# Autodesk Inventor assembly: KitBot-Obr
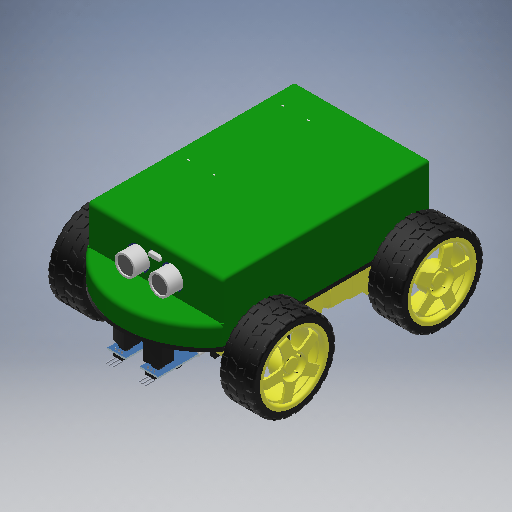
[picture p0: Inventor's stored thumbnail of the model, 512x512]
Saved by Autodesk Inventor 2025.1 (Build 291241020, 241B)
## iProperties
Created: 2024-12-26
Part Number: KitBot-Obr
Document SubType Name: Assembly
Designer: 53433618895
Author: 53433618895
## Documents named in this file (10)
- C:\Users\53433618895\OneDrive - SESISENAISP - Corporativo\FRC\2025\OBR\KitBot-Obr.iam
- C:\Users\53433618895\OneDrive - SESISENAISP - Corporativo\FRC\2025\OBR\tampa obr.ipt
- C:\Users\53433618895\OneDrive - SESISENAISP - Corporativo\FRC\2025\OBR\BASE.ipt
- C:\Users\53433618895\OneDrive - SESISENAISP - Corporativo\FRC\2025\OBR\arduino uno.iam
- C:\Users\53433618895\OneDrive - SESISENAISP - Corporativo\FRC\2025\OBR\Battery Holder ASSY V2.iam
- C:\Users\53433618895\OneDrive - SESISENAISP - Corporativo\FRC\2025\OBR\HCSR04 Ultrasonic Sensor.ipt
- C:\Users\53433618895\OneDrive - SESISENAISP - Corporativo\FRC\2025\OBR\infravermelho.ipt
- C:\Users\53433618895\OneDrive - SESISENAISP - Corporativo\FRC\2025\OBR\dc_motor_and_wheel.ipt
- C:\Users\53433618895\OneDrive - SESISENAISP - Corporativo\FRC\2025\OBR\Ponte H.ipt
- C:\Users\53433618895\OneDrive - SESISENAISP - Corporativo\FRC\2025\OBR\protobord.ipt
## Components (13 placed, 9 different names)
1. tampa obr:1 — Alinhado:1, Coincidente:10, Coincidente:26, Coincidente:27, Coincidente:28, Coincidente:40, Coincidente:41, Coincidente:43, Ângulo:1, Alinhado:13, Alinhado:14
2. BASE:1 — Alinhado:1, Coincidente:16, Coincidente:18, Alinhado:3, Coincidente:36, Coincidente:37, Alinhado:6, Rígida:1, Rígida:2, Coincidente:42, Alinhado:8, Alinhado:11, Alinhado:12, Coincidente:44, Alinhado:13, Alinhado:14
3. dc_motor_and_wheel:5 — Alinhado:12, Coincidente:44, Alinhado:15
4. HCSR04 Ultrasonic Sensor:1 — Coincidente:10
5. infravermelho:1 — Rígida:1
6. arduino uno:1 [sub-assembly] — Coincidente:26, Coincidente:27, Coincidente:28
7. infravermelho:2 — Rígida:2
8. Battery Holder ASSY V2:3 [sub-assembly] — Coincidente:40, Coincidente:41
9. protobord:1 — Coincidente:43, Ângulo:1
10. Ponte H:1 — Coincidente:42, Alinhado:8
11. dc_motor_and_wheel:4 — Coincidente:16, Coincidente:18, Alinhado:3
12. dc_motor_and_wheel:1 — Coincidente:36, Coincidente:37, Alinhado:6, Alinhado:9, Alinhado:10
13. dc_motor_and_wheel:3 — Alinhado:9, Alinhado:10, Alinhado:11, Alinhado:15
## Relationships (27: Mate 13, Flush 11, WeldJoint 2, Angle 1)
- Alinhado:1 [Flush]: tampa obr:1 ↔ BASE:1
- Coincidente:10 [Mate] (0.1 mm): tampa obr:1 ↔ HCSR04 Ultrasonic Sensor:1
- Coincidente:16 [Mate]: BASE:1 ↔ dc_motor_and_wheel:4
- Coincidente:18 [Mate]: BASE:1 ↔ dc_motor_and_wheel:4
- Alinhado:3 [Flush]: BASE:1 ↔ dc_motor_and_wheel:4
- Coincidente:26 [Mate]: tampa obr:1 ↔ arduino uno:1
- Coincidente:27 [Mate] (10 mm): tampa obr:1 ↔ arduino uno:1
- Coincidente:28 [Mate]: tampa obr:1 ↔ arduino uno:1
- Coincidente:36 [Mate]: BASE:1 ↔ dc_motor_and_wheel:1
- Coincidente:37 [Mate]: BASE:1 ↔ dc_motor_and_wheel:1
- Alinhado:6 [Flush]: BASE:1 ↔ dc_motor_and_wheel:1
- Rígida:1 [WeldJoint]: BASE:1 ↔ infravermelho:1
- Rígida:2 [WeldJoint]: BASE:1 ↔ infravermelho:2
- Coincidente:40 [Mate]: tampa obr:1 ↔ Battery Holder ASSY V2:3
- Coincidente:41 [Mate]: tampa obr:1 ↔ Battery Holder ASSY V2:3
- Coincidente:42 [Mate]: BASE:1 ↔ Ponte H:1
- Alinhado:8 [Flush] (25.4 mm): BASE:1 ↔ Ponte H:1
- Coincidente:43 [Mate]: tampa obr:1 ↔ protobord:1
- Ângulo:1 [Angle] (0 deg): tampa obr:1 ↔ protobord:1
- Alinhado:9 [Flush]: dc_motor_and_wheel:1 ↔ dc_motor_and_wheel:3
- Alinhado:10 [Flush]: dc_motor_and_wheel:1 ↔ dc_motor_and_wheel:3
- Alinhado:11 [Flush]: BASE:1 ↔ dc_motor_and_wheel:3
- Alinhado:12 [Flush]: BASE:1 ↔ dc_motor_and_wheel:5
- Coincidente:44 [Mate]: BASE:1 ↔ dc_motor_and_wheel:5
- Alinhado:13 [Flush]: tampa obr:1 ↔ BASE:1
- Alinhado:14 [Flush]: tampa obr:1 ↔ BASE:1
- Alinhado:15 [Flush]: dc_motor_and_wheel:5 ↔ dc_motor_and_wheel:3
